(part 1 of 2)
# Autodesk Inventor assembly: Ensamblaje SCARA
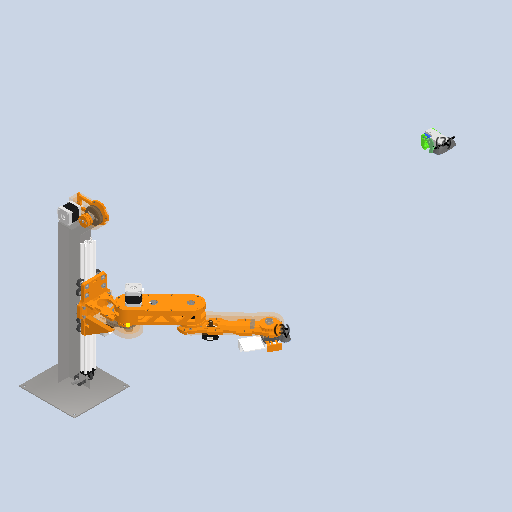
[picture p0: Inventor's stored thumbnail of the model, 512x512]
Saved by Autodesk Inventor 2026 (Build 300175050, 175E)
## iProperties
Created: 2025-07-17
Part Number: Ensamblaje SCARA
Document SubType Name: Assembly
Designer: bello
Mass: 5040.16 g
Surface Area: 9503.65 cm^2
Volume: 2049.58 cm^3
Density: 2.45911 g/cm^3
Author: bello
## Documents named in this file (71)
- A:\Federico Bellomi\UNLZ\5. Quinto Año\Proyecto Final\Ensamblaje\Ensamblaje SCARA.iam
- A:\Federico Bellomi\UNLZ\5. Quinto Año\Proyecto Final\Ensamblaje\Eje Z\Poste.ipt
- A:\Federico Bellomi\UNLZ\5. Quinto Año\Proyecto Final\Ensamblaje\Eje Z\Perfil 2040 200 mm v4.ipt
- A:\Federico Bellomi\UNLZ\5. Quinto Año\Proyecto Final\Ensamblaje\Eje Z\Tapa perfil de aluminio.ipt
- A:\Federico Bellomi\UNLZ\5. Quinto Año\Proyecto Final\Ensamblaje\download\Nema+17+Motor+Assembled\Nema+17+Motor+Assembled\Nema+17+Motor+Assembled.iam
- A:\Federico Bellomi\UNLZ\5. Quinto Año\Proyecto Final\Ensamblaje\Primer Segmento\Rueda v.ipt
- C:\Users\bello\OneDrive\Documentos\Inventor\Content Center Files\R2026\es-ES\DIN 625 SKF(1)\DIN 625 SKF - SKF 625-Z.ipt
- A:\Federico Bellomi\UNLZ\5. Quinto Año\Proyecto Final\Ensamblaje\download\Nema+17+Motor+Assembled\Engranaje para nema 17.ipt
- C:\Users\bello\OneDrive\Documentos\Inventor\Content Center Files\R2026\es-ES\DIN 625 SKF(1)\DIN 625 SKF - SKF 608-Z.ipt
- A:\Federico Bellomi\UNLZ\5. Quinto Año\Proyecto Final\Ensamblaje\Primer Segmento\Primer segmento - superior v1.2.ipt
- A:\Federico Bellomi\UNLZ\5. Quinto Año\Proyecto Final\Ensamblaje\Eje Z\Engranaje Insertado en pin.ipt
- C:\Users\bello\OneDrive\Documentos\Inventor\Content Center Files\R2026\es-ES\ISO 4014(2)\ISO 4014 - M5 x 35 - ISO.ipt
- C:\Users\bello\OneDrive\Documentos\Inventor\Content Center Files\R2026\es-ES\ISO 4014(2)\ISO 4014 - M8 x 50 - ISO.ipt
- C:\Users\bello\OneDrive\Documentos\Inventor\Content Center Files\R2026\es-ES\ISO 7089\ISO 7089 - 8 - 140 HV(1).ipt
- C:\Users\bello\OneDrive\Documentos\Inventor\Content Center Files\R2026\es-ES\ISO 7093 A\ISO 7093 A - ST 5 - 140 HV .ipt
- C:\Users\bello\OneDrive\Documentos\Inventor\Content Center Files\R2026\es-ES\ISO 4032(2)\ISO 4032 - M6 - ISO.ipt
- C:\Users\bello\OneDrive\Documentos\Inventor\Content Center Files\R2026\es-ES\ISO 4032(2)\ISO 4032 - M8 - ISO.ipt
- A:\Federico Bellomi\UNLZ\5. Quinto Año\Proyecto Final\Ensamblaje\Primer Segmento\Buje paraVslot.ipt
- C:\Users\bello\OneDrive\Documentos\Inventor\Content Center Files\R2026\es-ES\ISO 4032(2)\ISO 4032 - M5 - ISO.ipt
- A:\Federico Bellomi\UNLZ\5. Quinto Año\Proyecto Final\Ensamblaje\Eje Z\Buje para UPN.ipt
- C:\Users\bello\OneDrive\Documentos\Inventor\Content Center Files\R2026\es-ES\KS B 2023\KS B 2023 - 688 - 8 x 16 x 4 - 1.351.ipt
- A:\Federico Bellomi\UNLZ\5. Quinto Año\Proyecto Final\Ensamblaje\Primer Segmento\Soporte del primer segmento.ipt
- A:\Federico Bellomi\UNLZ\5. Quinto Año\Proyecto Final\Ensamblaje\Eje Z\Cono interno - Engranaje 1 eje Z.ipt
- A:\Federico Bellomi\UNLZ\5. Quinto Año\Proyecto Final\Ensamblaje\Eje Z\Engranaje 1 - Reductor Eje Z.ipt
- C:\Users\bello\OneDrive\Documentos\Inventor\Content Center Files\R2026\es-ES\BS 290 SKF(09)\BS 290 SKF - SKF 608-2Z.ipt
- C:\Users\bello\OneDrive\Documentos\Inventor\Content Center Files\R2026\es-ES\ISO 2338(2)\ISO 2338 - 8 h8 x 60.ipt
- C:\Users\bello\OneDrive\Documentos\Inventor\Content Center Files\R2026\es-ES\ISO 4032(2)\ISO 4032 - M3 - ISO.ipt
- A:\Federico Bellomi\UNLZ\5. Quinto Año\Proyecto Final\Ensamblaje\Eje Z\Caja reductora - eje z.ipt
- C:\Users\bello\OneDrive\Documentos\Inventor\Content Center Files\R2026\es-ES\ISO 4014(2)\ISO 4014 - M6 x 30 - ISO.ipt
- C:\Users\bello\OneDrive\Documentos\Inventor\Content Center Files\R2026\es-ES\ISO 7089\ISO 7089 - 6 - 140 HV(1).ipt
- A:\Federico Bellomi\UNLZ\5. Quinto Año\Proyecto Final\Ensamblaje\Eje Z\Tapa de caja reductora - eje z.ipt
- C:\Users\bello\OneDrive\Documentos\Inventor\Content Center Files\R2026\es-ES\ISO 4017(1)\ISO 4017 - M3 x 16 - ISO.ipt
- C:\Users\bello\OneDrive\Documentos\Inventor\Content Center Files\R2026\es-ES\ISO 7089\ISO 7089 - 3 - 140 HV(1).ipt
- A:\Federico Bellomi\UNLZ\5. Quinto Año\Proyecto Final\Ensamblaje\Eje Z\Engranaje 2 reductor Eje Z.ipt
- A:\Federico Bellomi\UNLZ\5. Quinto Año\Proyecto Final\Ensamblaje\Eje Z\Cono interno - Engranaje 2 eje Z.ipt
- A:\Federico Bellomi\UNLZ\5. Quinto Año\Proyecto Final\Ensamblaje\Primer Segmento\Engrajane doble - primer segmento.ipt
- A:\Federico Bellomi\UNLZ\5. Quinto Año\Proyecto Final\Ensamblaje\Primer Segmento\Engranaje simple - primer segmento.ipt
- A:\Federico Bellomi\UNLZ\5. Quinto Año\Proyecto Final\Ensamblaje\Primer Segmento\Segmento inferior.ipt
- C:\Users\bello\OneDrive\Documentos\Inventor\Content Center Files\R2026\es-ES\ISO 2338(2)\ISO 2338 - 8 h8 x 40.ipt
- A:\Federico Bellomi\UNLZ\5. Quinto Año\Proyecto Final\Ensamblaje\Primer Segmento\Polea Lisa - eje3mm.ipt
- C:\Users\bello\OneDrive\Documentos\Inventor\Content Center Files\R2026\es-ES\ISO 4014(2)\ISO 4014 - M3 x 20 - ISO.ipt
- C:\Users\bello\OneDrive\Documentos\Inventor\Content Center Files\R2026\es-ES\ISO 7045  H\ISO 7045 - M3 x 10_ - 4.8 - H - ISO.ipt
- C:\Users\bello\OneDrive\Documentos\Inventor\Content Center Files\R2026\es-ES\ISO 4017(1)\ISO 4017 - M5 x 25 - ISO.ipt
- C:\Users\bello\OneDrive\Documentos\Inventor\Content Center Files\R2026\es-ES\ISO 7089\ISO 7089 - 5 - 140 HV(1).ipt
- C:\Users\bello\OneDrive\Documentos\Inventor\Content Center Files\R2026\es-ES\JIS B 1521\JIS B 1521 - 6805 25x37x7x4.5.ipt
- C:\Users\bello\OneDrive\Documentos\Inventor\Content Center Files\R2026\es-ES\ISO 4017(1)\ISO 4017 - M4 x 40 - ISO.ipt
- C:\Users\bello\OneDrive\Documentos\Inventor\Content Center Files\R2026\es-ES\ISO 4032(2)\ISO 4032 - M4 - ISO.ipt
- C:\Users\bello\OneDrive\Documentos\Inventor\Content Center Files\R2026\es-ES\ISO 7045  H\ISO 7045 - M3 x 8_ - 4.8 - H - ISO.ipt
- A:\Federico Bellomi\UNLZ\5. Quinto Año\Proyecto Final\Ensamblaje\Segundo Segmento\Segundo segmento - superior.ipt
- A:\Federico Bellomi\UNLZ\5. Quinto Año\Proyecto Final\Ensamblaje\Segundo Segmento\Segundo segmento - inferior - Shape generator prueba 2 - 40%.ipt
- C:\Users\bello\OneDrive\Documentos\Inventor\Content Center Files\R2026\es-ES\ISO 7045  H\ISO 7045 - M4 x 16_ - 4.8 - H - ISO.ipt
- C:\Users\bello\OneDrive\Documentos\Inventor\Content Center Files\R2026\es-ES\ISO 7089\ISO 7089 - 4 - 140 HV(1).ipt
- A:\Federico Bellomi\UNLZ\5. Quinto Año\Proyecto Final\Ensamblaje\Segundo Segmento\Engranaje simple - segundo segmento.ipt
- A:\Federico Bellomi\UNLZ\5. Quinto Año\Proyecto Final\Ensamblaje\Segundo Segmento\Joint - Segundo segmento.ipt
- A:\Federico Bellomi\UNLZ\5. Quinto Año\Proyecto Final\Ensamblaje\Tercer Segmento\Tercer Segmento - inferior.ipt
- A:\Federico Bellomi\UNLZ\5. Quinto Año\Proyecto Final\Ensamblaje\Tercer Segmento\Tercer segmento - superior.ipt
- A:\Federico Bellomi\UNLZ\5. Quinto Año\Proyecto Final\Ensamblaje\Tercer Segmento\nema17_pancake\nema17_pancake\nema17_pancake.ipt
- A:\Federico Bellomi\UNLZ\5. Quinto Año\Proyecto Final\Ensamblaje\Primer Segmento\Joint - Primer segmento.ipt
- C:\Users\bello\OneDrive\Documentos\Inventor\Content Center Files\R2026\es-ES\ISO 2338(2)\ISO 2338 - 8 h8 x 50.ipt
- C:\Users\bello\OneDrive\Documentos\Inventor\Content Center Files\R2026\es-ES\ISO 2338(2)\ISO 2338 - 8 h8 x 30.ipt
- A:\Federico Bellomi\UNLZ\5. Quinto Año\Proyecto Final\Ensamblaje\Gripper\Base - Gripper.ipt
- A:\Federico Bellomi\UNLZ\5. Quinto Año\Proyecto Final\pince-robot-sg90-gripper-1.snapshot.26\Pince robot SG90\roue dentée 38A1\roue dentée 38A1\roue dentée 38A1.ipt
- A:\Federico Bellomi\UNLZ\5. Quinto Año\Proyecto Final\pince-robot-sg90-gripper-1.snapshot.26\Pince robot SG90\roue dentée 38B1\roue dentée 38B1\roue dentée 38B1.ipt
- A:\Federico Bellomi\UNLZ\5. Quinto Año\Proyecto Final\Ensamblaje\Gripper\Servo SG90\Servo SG90\Servo SG90.ipt
- A:\Federico Bellomi\UNLZ\5. Quinto Año\Proyecto Final\Ensamblaje\Gripper\logitech-c270-webcam-1.snapshot.1\Logitech c270\Logitech c270\Logitech c270.ipt
- A:\Federico Bellomi\UNLZ\5. Quinto Año\Proyecto Final\Ensamblaje\Gripper\Base - version 2.ipt
- A:\Federico Bellomi\UNLZ\5. Quinto Año\Proyecto Final\Ensamblaje\Gripper\logitech-c270-webcam-1.snapshot.1\Logitech c270\Round_gear.ipt
- A:\Federico Bellomi\UNLZ\5. Quinto Año\Proyecto Final\Ensamblaje\Gripper\Tapa - Gripper.ipt
- A:\Federico Bellomi\UNLZ\5. Quinto Año\Proyecto Final\Ensamblaje\Gripper\Pata Izquierda - versión 3.ipt
- A:\Federico Bellomi\UNLZ\5. Quinto Año\Proyecto Final\Ensamblaje\Gripper\Pata derecha - versión 3.ipt
- A:\Federico Bellomi\UNLZ\5. Quinto Año\Proyecto Final\Ensamblaje\Gripper\Base Marcador ECU + Gripper.ipt
## Components (260 placed, 70 different names)
1. Poste:1 — Coincidencia:1, Nivelación:1, Coincidencia:287, Coincidencia:288, Coincidencia:290, Coincidencia:484, Ángulo:3, Coincidencia:507, Ángulo:4, Coincidencia:508, Coincidencia:515, Ángulo:28, Ángulo:29
2. Perfil 2040 200 mm v4:2 — Insertar:1, Insertar:2, Coincidencia:424
3. Perfil 2040 200 mm v4:3 — Insertar:1, Coincidencia:1, Nivelación:1, Insertar:2, Coincidencia:1235, Nivelación:138
4. Rueda v:9
5. DIN 625 SKF- con escudo Z SKF 625-Z:18
6. DIN 625 SKF- con escudo Z SKF 625-Z:19
7. ISO 4014 M5 x 35:1 — Coincidencia:137, Coincidencia:138, Coincidencia:142, Coincidencia:143
8. ISO 7093 A ST 5 - 140 HV - A:1 — Coincidencia:138, Coincidencia:144
9. ISO 7093 A ST 5 - 140 HV - A:2 — Coincidencia:137, Coincidencia:142
10. ISO 4032 M6:1 — Coincidencia:143, Coincidencia:144
11. ISO 4014 M8 x 50:1 — Coincidencia:282, Coincidencia:283, Coincidencia:287, Coincidencia:289, Coincidencia:295, Coincidencia:297, Coincidencia:299
12. ISO 7089 8:1 — Coincidencia:282, Coincidencia:283, Coincidencia:288
13. ISO 7089 8:2 — Coincidencia:289, Coincidencia:290, Coincidencia:298
14. Buje para UPN:1 — Coincidencia:296, Coincidencia:297, Coincidencia:298
15. ISO 4032 M8:1 — Coincidencia:299, Coincidencia:300
16. KS B 2023 688 - 8 x 16 x 4:3 — Coincidencia:292, Coincidencia:293, Coincidencia:296
17. Engranaje Insertado en pin:1 — Coincidencia:291, Coincidencia:292, Coincidencia:293, Coincidencia:294, Coincidencia:295
18. KS B 2023 688 - 8 x 16 x 4:4 — Coincidencia:291, Coincidencia:294, Coincidencia:300
19. Tapa perfil de aluminio:1 — Coincidencia:424
20. ISO 2338 8 h8 x 60:1 — Coincidencia:469, Nivelación:62, Coincidencia:536, Coincidencia:551
21. BS 290 SKF- con dos escudos Z SKF 608-2Z:3 — Coincidencia:467, Coincidencia:469, Coincidencia:518, Nivelación:70
22. BS 290 SKF- con dos escudos Z SKF 608-2Z:4 — Coincidencia:467, Nivelación:62, Coincidencia:490, Nivelación:65, Coincidencia:537
23. Nema+17+Motor+Assembled:2 [sub-assembly] — Ángulo:3, Coincidencia:516, Coincidencia:517
24. ISO 4014 M6 x 30:1 — Nivelación:63, Coincidencia:509, Coincidencia:511, Coincidencia:514
25. ISO 4014 M6 x 30:2 — Nivelación:63, Coincidencia:481, Coincidencia:482, Coincidencia:510
26. ISO 4032 M6:2 — Coincidencia:481, Coincidencia:487
27. ISO 7089 6:2 — Coincidencia:482, Coincidencia:484, Coincidencia:487
28. Tapa de caja reductora - eje z:1 — Coincidencia:490, Nivelación:65, Coincidencia:519, Coincidencia:694, Coincidencia:695, Coincidencia:696, Coincidencia:697, Coincidencia:698, Coincidencia:699, Coincidencia:700, Coincidencia:701
29. ISO 4032 M6:3 — Coincidencia:512, Coincidencia:513
30. ISO 7089 6:3 — Coincidencia:512, Coincidencia:513, Coincidencia:514, Coincidencia:515
31. Caja reductora - eje z:1 — Coincidencia:507, Ángulo:4, Coincidencia:508, Coincidencia:509, Coincidencia:510, Coincidencia:511, Coincidencia:516, Coincidencia:517, Coincidencia:518, Nivelación:70, Coincidencia:519, Coincidencia:552
32. Engranaje 1 - Reductor Eje Z:2
33. Cono interno - Engranaje 1 eje Z:2 — Coincidencia:536, Coincidencia:537
34. ISO 4032 M3:3
35. ISO 4032 M3:4
36. ISO 4017 M3 x 16:3
37. ISO 4017 M3 x 16:4
38. ISO 7089 3:3
39. ISO 7089 3:4
40. Engranaje 2 reductor Eje Z:1 — Coincidencia:538, Coincidencia:539, Coincidencia:540, Coincidencia:541, Nivelación:78, Coincidencia:542, Nivelación:79, Ángulo:5, Ángulo:6
41. Cono interno - Engranaje 2 eje Z:1 — Coincidencia:538, Coincidencia:539, Coincidencia:540, Coincidencia:543, Coincidencia:545, Coincidencia:547, Coincidencia:549, Coincidencia:551, Coincidencia:552
42. ISO 4017 M3 x 16:5 — Coincidencia:543, Coincidencia:544, Coincidencia:550
43. ISO 7089 3:5 — Coincidencia:544, Coincidencia:549, Coincidencia:550
44. ISO 4032 M3:5 — Coincidencia:541, Nivelación:78, Ángulo:5
45. ISO 4032 M3:6 — Coincidencia:542, Nivelación:79, Ángulo:6
46. ISO 7089 3:6 — Coincidencia:546, Coincidencia:547, Coincidencia:548
47. ISO 4017 M3 x 16:6 — Coincidencia:545, Coincidencia:546, Coincidencia:548
48. ISO 7045 H M3 x 10 - 4.8 - H:1 — Coincidencia:697, Coincidencia:699
49. ISO 7045 H M3 x 10 - 4.8 - H:2 — Coincidencia:695, Coincidencia:700
50. ISO 7045 H M3 x 10 - 4.8 - H:3 — Coincidencia:696, Coincidencia:698
51. ISO 7045 H M3 x 10 - 4.8 - H:4 — Coincidencia:694, Coincidencia:701
52. ISO 2338 8 h8 x 40:3 — Coincidencia:901, Nivelación:110, Coincidencia:917
53. DIN 625 SKF- con escudo Z SKF 608-Z:5 — Coincidencia:895, Nivelación:107, Coincidencia:897
54. Engrajane doble - primer segmento:2 — Coincidencia:917, Nivelación:113, Nivelación:114
55. DIN 625 SKF- con escudo Z SKF 608-Z:6 — Coincidencia:899, Nivelación:108, Coincidencia:901, Nivelación:110
56. DIN 625 SKF- con escudo Z SKF 608-Z:9 — Coincidencia:900, Nivelación:109, Coincidencia:1197, Nivelación:133
57. Rueda v:28
58. DIN 625 SKF- con escudo Z SKF 625-Z:56
59. DIN 625 SKF- con escudo Z SKF 625-Z:57
60. ISO 4014 M5 x 35:21
61. Buje paraVslot:20
62. Rueda v:29
63. DIN 625 SKF- con escudo Z SKF 625-Z:58
64. DIN 625 SKF- con escudo Z SKF 625-Z:59
65. ISO 4014 M5 x 35:22
66. Buje paraVslot:21
67. ISO 4032 M5:22
68. ISO 7093 A ST 5 - 140 HV - A:28
69. ISO 4032 M5:23
70. ISO 7093 A ST 5 - 140 HV - A:29
71. Soporte del primer segmento:2 — Coincidencia:881, Coincidencia:882, Coincidencia:883, Coincidencia:884, Coincidencia:885, Coincidencia:886, Coincidencia:888, Ángulo:29, Coincidencia:1235, Nivelación:138
72. ISO 7093 A ST 5 - 140 HV - A:30
73. ISO 7093 A ST 5 - 140 HV - A:31
74. Rueda v:30
75. DIN 625 SKF- con escudo Z SKF 625-Z:60
76. DIN 625 SKF- con escudo Z SKF 625-Z:61
77. ISO 4014 M5 x 35:23
78. Buje paraVslot:22
79. ISO 4032 M5:24
80. ISO 7093 A ST 5 - 140 HV - A:32
81. ISO 7093 A ST 5 - 140 HV - A:33
82. Rueda v:31
83. DIN 625 SKF- con escudo Z SKF 625-Z:62
84. DIN 625 SKF- con escudo Z SKF 625-Z:63
85. ISO 4014 M5 x 35:24
86. Buje paraVslot:23
87. ISO 4032 M5:25
88. ISO 7093 A ST 5 - 140 HV - A:34
89. ISO 7093 A ST 5 - 140 HV - A:35
90. Engranaje para nema 17:4 — Coincidencia:903, Nivelación:114
91. Rueda v:32
92. DIN 625 SKF- con escudo Z SKF 625-Z:64
93. DIN 625 SKF- con escudo Z SKF 625-Z:65
94. ISO 4014 M5 x 35:25
95. Buje paraVslot:24
96. ISO 4032 M5:26
97. ISO 7093 A ST 5 - 140 HV - A:36
98. Rueda v:33
99. DIN 625 SKF- con escudo Z SKF 625-Z:66
100. DIN 625 SKF- con escudo Z SKF 625-Z:67
101. ISO 4014 M5 x 35:26
102. Buje paraVslot:25
103. ISO 4032 M5:27
104. ISO 7093 A ST 5 - 140 HV - A:37
105. Rueda v:34
106. DIN 625 SKF- con escudo Z SKF 625-Z:68
107. DIN 625 SKF- con escudo Z SKF 625-Z:69
108. ISO 4014 M5 x 35:27
109. Buje paraVslot:26
110. ISO 4032 M5:28
111. ISO 7093 A ST 5 - 140 HV - A:38
112. Rueda v:35
113. DIN 625 SKF- con escudo Z SKF 625-Z:70
114. DIN 625 SKF- con escudo Z SKF 625-Z:71
115. ISO 4014 M5 x 35:28
116. Buje paraVslot:27
117. ISO 4032 M5:29
118. ISO 7093 A ST 5 - 140 HV - A:39
119. ISO 4017 M5 x 25:5 — Coincidencia:884, Coincidencia:887, Ángulo:24
120. ISO 4017 M5 x 25:6 — Coincidencia:886, Ángulo:26, Coincidencia:890
121. ISO 4017 M5 x 25:7 — Coincidencia:885, Ángulo:27, Coincidencia:889
122. ISO 4017 M5 x 25:8 — Coincidencia:883, Ángulo:25, Coincidencia:891
123. ISO 4032 M5:30
124. ISO 4032 M5:31
125. ISO 4032 M5:32
126. ISO 4032 M5:33
127. ISO 7089 5:5
128. ISO 7089 5:6
129. ISO 7089 5:7
130. ISO 7089 5:8
131. Segmento inferior:1 — Coincidencia:881, Coincidencia:882, Coincidencia:887, Ángulo:24, Ángulo:25, Coincidencia:888, Ángulo:26, Ángulo:27, Coincidencia:889, Coincidencia:890, Coincidencia:891, Ángulo:28, Coincidencia:892, Coincidencia:893, Coincidencia:894, Coincidencia:895, Nivelación:107, Coincidencia:896, Coincidencia:898, Coincidencia:900, Nivelación:109
132. Nema+17+Motor+Assembled:5 [sub-assembly] — Coincidencia:892, Coincidencia:893, Coincidencia:894, Coincidencia:903
133. Primer segmento - superior v1.2:1 — Coincidencia:896, Coincidencia:897, Coincidencia:898, Coincidencia:899, Nivelación:108, Coincidencia:904, Coincidencia:905, Coincidencia:906, Coincidencia:907, Coincidencia:908, Coincidencia:909, Coincidencia:910, Coincidencia:911, Coincidencia:912, Coincidencia:913, Coincidencia:914, Coincidencia:915, Coincidencia:916, Nivelación:112, Coincidencia:1039, Coincidencia:1041
134. JIS B 1521 6805 25x37x7:3 — Coincidencia:916, Nivelación:112, Coincidencia:919
135. Engranaje simple - primer segmento:1 — Coincidencia:919, Nivelación:113, Coincidencia:929, Coincidencia:930, Coincidencia:931, Coincidencia:932, Coincidencia:1042, Coincidencia:1043, Coincidencia:1044, Coincidencia:1045
136. ISO 4017 M4 x 40:1 — Coincidencia:931, Coincidencia:935, Coincidencia:1043
137. ISO 4017 M4 x 40:2 — Coincidencia:930, Coincidencia:934, Coincidencia:1042
138. ISO 4017 M4 x 40:3 — Coincidencia:932, Coincidencia:936, Coincidencia:1045, Coincidencia:1184
139. ISO 4017 M4 x 40:4 — Coincidencia:929, Coincidencia:933, Coincidencia:1044
140. ISO 7045 H M3 x 8 - 4.8 - H:14 — Coincidencia:904, Coincidencia:910
141. ISO 7045 H M3 x 8 - 4.8 - H:15 — Coincidencia:909, Coincidencia:911
142. ISO 4032 M4:1 — Coincidencia:935, Coincidencia:1046
143. ISO 4032 M4:2 — Coincidencia:936, Coincidencia:1048
144. ISO 4032 M4:3 — Coincidencia:933, Coincidencia:1049
145. ISO 4032 M4:4 — Coincidencia:934, Coincidencia:1047
146. ISO 7045 H M3 x 8 - 4.8 - H:16 — Coincidencia:905, Coincidencia:912
147. ISO 7045 H M3 x 8 - 4.8 - H:17 — Coincidencia:908, Coincidencia:915
148. ISO 7045 H M3 x 8 - 4.8 - H:18 — Coincidencia:906, Coincidencia:913
149. ISO 7045 H M3 x 8 - 4.8 - H:19 — Coincidencia:907, Coincidencia:914
150. Segundo segmento - inferior - Shape generator prueba 2 - 40%:1 — Coincidencia:944, Coincidencia:945, Coincidencia:946, Coincidencia:947, Coincidencia:948, Coincidencia:949, Coincidencia:962, Coincidencia:963, Coincidencia:964, Coincidencia:965, Coincidencia:966, Coincidencia:967, Coincidencia:980, Coincidencia:981, Coincidencia:982, Nivelación:122, Coincidencia:1016, Coincidencia:1038, Coincidencia:1040, Coincidencia:1041, Coincidencia:1063, Coincidencia:1143, Coincidencia:1144, Coincidencia:1145, Coincidencia:1233, Coincidencia:1234
151. ISO 7045 H M4 x 16 - 4.8 - H:1 — Coincidencia:947, Coincidencia:958, Coincidencia:971, Coincidencia:1053, Coincidencia:1057
152. ISO 7045 H M4 x 16 - 4.8 - H:2 — Coincidencia:948, Coincidencia:961, Coincidencia:972, Coincidencia:1052, Coincidencia:1061
153. ISO 7045 H M4 x 16 - 4.8 - H:3 — Coincidencia:946, Coincidencia:957, Coincidencia:970, Coincidencia:1051, Coincidencia:1058
154. ISO 7045 H M4 x 16 - 4.8 - H:4 — Coincidencia:944, Coincidencia:955, Coincidencia:969, Coincidencia:1054, Coincidencia:1059
155. ISO 7045 H M4 x 16 - 4.8 - H:5 — Coincidencia:945, Coincidencia:956, Coincidencia:968, Coincidencia:1055, Coincidencia:1060
156. ISO 7045 H M4 x 16 - 4.8 - H:6 — Coincidencia:949, Coincidencia:959, Coincidencia:973, Coincidencia:1050, Coincidencia:1056
157. ISO 4032 M4:5 — Coincidencia:968, Coincidencia:977
158. ISO 4032 M4:6 — Coincidencia:969, Coincidencia:978
159. ISO 4032 M4:7 — Coincidencia:970, Coincidencia:975
160. ISO 4032 M4:8 — Coincidencia:971, Coincidencia:979
161. ISO 7089 4:1 — Coincidencia:957, Coincidencia:964
162. ISO 7089 4:2 — Coincidencia:955, Coincidencia:967, Coincidencia:978
163. ISO 7089 4:3 — Coincidencia:956, Coincidencia:966, Coincidencia:977
164. ISO 7089 4:4 — Coincidencia:958, Coincidencia:965, Coincidencia:975, Coincidencia:979
165. ISO 7089 4:5 — Coincidencia:959, Coincidencia:962
166. ISO 7089 4:6 — Coincidencia:961, Coincidencia:963, Coincidencia:974, Coincidencia:976
167. ISO 4032 M4:9 — Coincidencia:972, Coincidencia:976
168. ISO 4032 M4:10 — Coincidencia:973, Coincidencia:974
169. Segundo segmento - superior:1 — Coincidencia:980, Coincidencia:981, Coincidencia:982, Coincidencia:983, Coincidencia:984, Coincidencia:985, Coincidencia:987, Nivelación:115, Coincidencia:988, Nivelación:116, Coincidencia:1000, Coincidencia:1001, Coincidencia:1002, Coincidencia:1003, Coincidencia:1004, Coincidencia:1005, Coincidencia:1006, Coincidencia:1007, Coincidencia:1008, Coincidencia:1009, Coincidencia:1010, Coincidencia:1011, Coincidencia:1012, Coincidencia:1013, Coincidencia:1014, Coincidencia:1015, Coincidencia:1062
170. Engranaje para nema 17:5 — Coincidencia:986, Nivelación:119
171. DIN 625 SKF- con escudo Z SKF 608-Z:10 — Coincidencia:987, Nivelación:115, Coincidencia:989, Nivelación:117
172. DIN 625 SKF- con escudo Z SKF 608-Z:11 — Coincidencia:988, Nivelación:116, Coincidencia:1198, Nivelación:134
173. Engrajane doble - primer segmento:3 — Coincidencia:990, Nivelación:119, Nivelación:123
174. ISO 2338 8 h8 x 40:4 — Coincidencia:989, Nivelación:117, Coincidencia:990
175. Nema+17+Motor+Assembled:6 [sub-assembly] — Coincidencia:983, Coincidencia:984, Coincidencia:985, Coincidencia:986
176. ISO 4017 M4 x 40:5 — Coincidencia:1025, Coincidencia:1071, Coincidencia:1078
177. ISO 4017 M4 x 40:6 — Coincidencia:1027, Coincidencia:1073, Coincidencia:1076
178. ISO 4017 M4 x 40:7 — Coincidencia:1024, Coincidencia:1074, Coincidencia:1077
179. ISO 4017 M4 x 40:8 — Coincidencia:1026, Coincidencia:1072, Coincidencia:1075
180. Engranaje simple - segundo segmento:1 — Coincidencia:1024, Coincidencia:1025, Coincidencia:1026, Coincidencia:1027, Nivelación:123, Coincidencia:1064, Coincidencia:1066, Coincidencia:1067
181. ISO 7045 H M3 x 8 - 4.8 - H:20 — Coincidencia:1000, Coincidencia:1013
182. ISO 7045 H M3 x 8 - 4.8 - H:21 — Coincidencia:1001, Coincidencia:1014
183. ISO 7045 H M3 x 8 - 4.8 - H:22 — Coincidencia:1002, Coincidencia:1009
184. ISO 7045 H M3 x 8 - 4.8 - H:23 — Coincidencia:1003, Coincidencia:1012
185. ISO 7045 H M3 x 8 - 4.8 - H:24 — Coincidencia:1004, Coincidencia:1011
186. ISO 7045 H M3 x 8 - 4.8 - H:25 — Coincidencia:1007, Coincidencia:1015
187. ISO 7045 H M3 x 8 - 4.8 - H:26 — Coincidencia:1006, Coincidencia:1008
188. ISO 7045 H M3 x 8 - 4.8 - H:27 — Coincidencia:1005, Coincidencia:1010
189. DIN 625 SKF- con escudo Z SKF 608-Z:12 — Nivelación:122, Coincidencia:1016
190. Tercer Segmento - inferior:1 — Coincidencia:1031, Coincidencia:1032, Coincidencia:1033, Coincidencia:1035, Coincidencia:1036, Coincidencia:1037, Coincidencia:1127, Coincidencia:1160, Coincidencia:1161, Coincidencia:1162, Nivelación:127, Coincidencia:1165, Coincidencia:1166, Ángulo:30, Coincidencia:1167, Coincidencia:1168, Coincidencia:1169, Coincidencia:1170, Coincidencia:1171, Coincidencia:1172, Coincidencia:1173, Coincidencia:1174, Coincidencia:1175, Coincidencia:1176, Coincidencia:1177, Coincidencia:1178, Coincidencia:1179, Coincidencia:1180, Coincidencia:1181, Coincidencia:1182, Coincidencia:1183, Coincidencia:1237
191. Tercer segmento - superior:1 — Coincidencia:1031, Coincidencia:1032, Coincidencia:1033, Coincidencia:1068, Coincidencia:1069, Coincidencia:1070, Coincidencia:1111, Coincidencia:1113, Coincidencia:1114, Coincidencia:1115, Coincidencia:1116, Coincidencia:1117, Coincidencia:1127, Coincidencia:1191, Nivelación:131
192. nema17_pancake:1 — Coincidencia:1035, Coincidencia:1036, Coincidencia:1037, Coincidencia:1126
193. Joint - Primer segmento:1 — Coincidencia:1038, Coincidencia:1039, Coincidencia:1040, Coincidencia:1046, Coincidencia:1047, Coincidencia:1048, Coincidencia:1049, Coincidencia:1050, Coincidencia:1051, Coincidencia:1052, Coincidencia:1053, Coincidencia:1054, Coincidencia:1055, Coincidencia:1056, Coincidencia:1057, Coincidencia:1058, Coincidencia:1059, Coincidencia:1060, Coincidencia:1061, Coincidencia:1184
194. JIS B 1521 6805 25x37x7:5 — Coincidencia:1062, Coincidencia:1063, Coincidencia:1064, Coincidencia:1065
195. Joint - Segundo segmento:1 — Coincidencia:1065, Coincidencia:1066, Coincidencia:1067, Coincidencia:1068, Coincidencia:1069, Coincidencia:1070, Coincidencia:1075, Coincidencia:1076, Coincidencia:1077, Coincidencia:1078, Coincidencia:1079, Coincidencia:1080, Coincidencia:1081, Coincidencia:1082, Coincidencia:1095, Coincidencia:1096, Coincidencia:1097, Coincidencia:1098, Coincidencia:1103, Coincidencia:1104, Coincidencia:1105, Coincidencia:1106, Coincidencia:1107, Coincidencia:1108, Coincidencia:1109, Coincidencia:1110
196. ISO 4032 M4:11 — Coincidencia:1073, Coincidencia:1081
197. ISO 4032 M4:12 — Coincidencia:1074, Coincidencia:1082
198. ISO 4032 M4:13 — Coincidencia:1072, Coincidencia:1079
199. ISO 4032 M4:14 — Coincidencia:1071, Coincidencia:1080
200. ISO 7045 H M4 x 16 - 4.8 - H:7 — Coincidencia:1098, Coincidencia:1105
201. ISO 7089 4:7 — Coincidencia:1114, Coincidencia:1120
202. ISO 4032 M4:15 — Coincidencia:1120
203. ISO 7045 H M4 x 16 - 4.8 - H:8 — Coincidencia:1097, Coincidencia:1106
204. ISO 7089 4:8 — Coincidencia:1115, Coincidencia:1119
205. ISO 4032 M4:16 — Coincidencia:1119
206. ISO 7045 H M4 x 16 - 4.8 - H:10 — Coincidencia:1104, Coincidencia:1110
207. ISO 7089 4:10 — Coincidencia:1111, Coincidencia:1112
208. ISO 4032 M4:18 — Coincidencia:1112
209. ISO 7045 H M4 x 16 - 4.8 - H:11 — Coincidencia:1096, Coincidencia:1108
210. ISO 7089 4:11 — Coincidencia:1116, Coincidencia:1118, Coincidencia:1122
211. ISO 4032 M4:19 — Coincidencia:1122
212. ISO 7045 H M4 x 16 - 4.8 - H:12 — Coincidencia:1095, Coincidencia:1107
213. ISO 7089 4:12 — Coincidencia:1117
214. ISO 4032 M4:20 — Coincidencia:1118
215. ISO 7045 H M4 x 16 - 4.8 - H:14 — Coincidencia:1103, Coincidencia:1109
216. ISO 7089 4:14 — Coincidencia:1113, Coincidencia:1121
217. ISO 4032 M4:22 — Coincidencia:1121
218. Engranaje para nema 17:6 — Coincidencia:1126, Nivelación:128
219. ISO 4014 M3 x 20:3 — Coincidencia:1233
220. Polea Lisa - eje3mm:3
221. ISO 4032 M3:11
222. ISO 4032 M3:12 — Coincidencia:1144
223. ISO 7089 3:9 — Coincidencia:1143, Coincidencia:1145, Coincidencia:1234
224. ISO 4014 M3 x 20:4 — Coincidencia:1160
225. Polea Lisa - eje3mm:4 — Nivelación:126
226. ISO 4032 M3:13
227. ISO 4032 M3:14 — Coincidencia:1167
228. ISO 7089 3:10 — Coincidencia:1165, Coincidencia:1237
229. ISO 4014 M3 x 20:5 — Coincidencia:1161
230. Polea Lisa - eje3mm:5 — Nivelación:126
231. ISO 4032 M3:15
232. ISO 4032 M3:16 — Coincidencia:1166, Ángulo:30
233. ISO 7089 3:11
234. Engranaje simple - segundo segmento:2 — Coincidencia:1163, Coincidencia:1164, Nivelación:128, Coincidencia:1222, Coincidencia:1223, Coincidencia:1236
235. JIS B 1521 6805 25x37x7:6 — Coincidencia:1162, Nivelación:127, Coincidencia:1163, Coincidencia:1164
236. ISO 7045 H M3 x 8 - 4.8 - H:28 — Coincidencia:1168, Coincidencia:1182
237. ISO 7045 H M3 x 8 - 4.8 - H:29 — Coincidencia:1169, Coincidencia:1180
238. ISO 7045 H M3 x 8 - 4.8 - H:30 — Coincidencia:1170, Coincidencia:1178
239. ISO 7045 H M3 x 8 - 4.8 - H:31 — Coincidencia:1171, Coincidencia:1176
240. ISO 7045 H M3 x 8 - 4.8 - H:32 — Coincidencia:1174, Coincidencia:1181
241. ISO 7045 H M3 x 8 - 4.8 - H:33 — Coincidencia:1175, Coincidencia:1183
242. ISO 7045 H M3 x 8 - 4.8 - H:34 — Coincidencia:1173, Coincidencia:1179
243. ISO 7045 H M3 x 8 - 4.8 - H:35 — Coincidencia:1172, Coincidencia:1177
244. DIN 625 SKF- con escudo Z SKF 608-Z:13 — Coincidencia:1191, Nivelación:131, Coincidencia:1199, Nivelación:135
245. ISO 2338 8 h8 x 50:1 — Coincidencia:1197, Nivelación:133
246. ISO 2338 8 h8 x 50:2 — Coincidencia:1198, Nivelación:134
247. ISO 2338 8 h8 x 30:1 — Coincidencia:1199, Nivelación:135
248. roue dentée 38A1:1 — Coincidencia:1213, Nivelación:136
249. roue dentée 38B1:1 — Coincidencia:1210
250. Base - Gripper:1 — Coincidencia:1207, Coincidencia:1208, Coincidencia:1209, Coincidencia:1210, Coincidencia:1211, Coincidencia:1212
251. Servo SG90:1 — Coincidencia:1207, Coincidencia:1208, Coincidencia:1209, Coincidencia:1213, Nivelación:136
252. Logitech c270:1 — Coincidencia:1211, Coincidencia:1212
253. Base - version 2:1 — Coincidencia:1214, Ángulo:31, Coincidencia:1215, Coincidencia:1217, Ángulo:32, Coincidencia:1218, Coincidencia:1219, Coincidencia:1220, Coincidencia:1221, Coincidencia:1228, Coincidencia:1229, Coincidencia:1230, Coincidencia:1231
254. Round_gear:1 — Coincidencia:1216, Nivelación:137
255. Servo SG90:2 — Coincidencia:1214, Ángulo:31, Coincidencia:1215, Coincidencia:1216, Nivelación:137
256. Logitech c270:2 — Coincidencia:1217, Ángulo:32, Coincidencia:1218
257. Tapa - Gripper:1 — Coincidencia:1219, Coincidencia:1220, Coincidencia:1221, Coincidencia:1222, Coincidencia:1223, Coincidencia:1236
258. Pata derecha - versión 3:1 — Coincidencia:1228, Coincidencia:1229
259. Pata Izquierda - versión 3:1 — Coincidencia:1230, Coincidencia:1231, Coincidencia:1232, Ángulo:33
260. Base Marcador ECU + Gripper:1 — Coincidencia:1232, Ángulo:33
## Relationships (552: Mate 480, Flush 52, Angle 18, Insert 2)
- Insertar:1: Perfil 2040 200 mm v4:2 ↔ Perfil 2040 200 mm v4:3
- Coincidencia:1 [Mate]: Poste:1 ↔ Perfil 2040 200 mm v4:3
- Nivelación:1 [Flush]: Poste:1 ↔ Perfil 2040 200 mm v4:3
- Insertar:2: Perfil 2040 200 mm v4:2 ↔ Perfil 2040 200 mm v4:3
- [Mate]: Rueda v:9 ↔ DIN 625 SKF- con escudo Z SKF 625-Z:18
- [Mate]: Rueda v:9 ↔ DIN 625 SKF- con escudo Z SKF 625-Z:19
- [Flush]: Rueda v:9 ↔ DIN 625 SKF- con escudo Z SKF 625-Z:18
- [Flush]: Rueda v:9 ↔ DIN 625 SKF- con escudo Z SKF 625-Z:19
- Coincidencia:137 [Mate]: ISO 4014 M5 x 35:1 ↔ ISO 7093 A ST 5 - 140 HV - A:2
- Coincidencia:138 [Mate]: ISO 4014 M5 x 35:1 ↔ ISO 7093 A ST 5 - 140 HV - A:1
- Coincidencia:142 [Mate]: ISO 4014 M5 x 35:1 ↔ ISO 7093 A ST 5 - 140 HV - A:2
- Coincidencia:143 [Mate]: ISO 4014 M5 x 35:1 ↔ ISO 4032 M6:1
- Coincidencia:144 [Mate]: ISO 7093 A ST 5 - 140 HV - A:1 ↔ ISO 4032 M6:1
- Coincidencia:282 [Mate]: ISO 4014 M8 x 50:1 ↔ ISO 7089 8:1
- Coincidencia:283 [Mate]: ISO 4014 M8 x 50:1 ↔ ISO 7089 8:1
- Coincidencia:287 [Mate]: Poste:1 ↔ ISO 4014 M8 x 50:1
- Coincidencia:288 [Mate]: Poste:1 ↔ ISO 7089 8:1
- Coincidencia:289 [Mate]: ISO 4014 M8 x 50:1 ↔ ISO 7089 8:2
- Coincidencia:290 [Mate]: Poste:1 ↔ ISO 7089 8:2
- Coincidencia:291 [Mate]: Engranaje Insertado en pin:1 ↔ KS B 2023 688 - 8 x 16 x 4:4
- Coincidencia:292 [Mate]: KS B 2023 688 - 8 x 16 x 4:3 ↔ Engranaje Insertado en pin:1
- Coincidencia:293 [Mate]: KS B 2023 688 - 8 x 16 x 4:3 ↔ Engranaje Insertado en pin:1
- Coincidencia:294 [Mate]: Engranaje Insertado en pin:1 ↔ KS B 2023 688 - 8 x 16 x 4:4
- Coincidencia:295 [Mate]: ISO 4014 M8 x 50:1 ↔ Engranaje Insertado en pin:1
- Coincidencia:296 [Mate]: Buje para UPN:1 ↔ KS B 2023 688 - 8 x 16 x 4:3
- Coincidencia:297 [Mate]: ISO 4014 M8 x 50:1 ↔ Buje para UPN:1
- Coincidencia:298 [Mate]: ISO 7089 8:2 ↔ Buje para UPN:1
- Coincidencia:299 [Mate]: ISO 4014 M8 x 50:1 ↔ ISO 4032 M8:1
- Coincidencia:300 [Mate]: ISO 4032 M8:1 ↔ KS B 2023 688 - 8 x 16 x 4:4
- Coincidencia:424 [Mate]: Perfil 2040 200 mm v4:2 ↔ Tapa perfil de aluminio:1
- Coincidencia:467 [Mate]: BS 290 SKF- con dos escudos Z SKF 608-2Z:3 ↔ BS 290 SKF- con dos escudos Z SKF 608-2Z:4
- Coincidencia:469 [Mate]: ISO 2338 8 h8 x 60:1 ↔ BS 290 SKF- con dos escudos Z SKF 608-2Z:3
- Nivelación:62 [Flush]: ISO 2338 8 h8 x 60:1 ↔ BS 290 SKF- con dos escudos Z SKF 608-2Z:4
- Nivelación:63 [Flush]: ISO 4014 M6 x 30:1 ↔ ISO 4014 M6 x 30:2
- Coincidencia:481 [Mate]: ISO 4014 M6 x 30:2 ↔ ISO 4032 M6:2
- Coincidencia:482 [Mate]: ISO 4014 M6 x 30:2 ↔ ISO 7089 6:2
- Coincidencia:484 [Mate]: Poste:1 ↔ ISO 7089 6:2
- Coincidencia:487 [Mate]: ISO 4032 M6:2 ↔ ISO 7089 6:2
- Coincidencia:490 [Mate]: BS 290 SKF- con dos escudos Z SKF 608-2Z:4 ↔ Tapa de caja reductora - eje z:1
- Ángulo:3 [Angle] (0 deg): Poste:1 ↔ Nema+17+Motor+Assembled:2
- Nivelación:65 [Flush]: BS 290 SKF- con dos escudos Z SKF 608-2Z:4 ↔ Tapa de caja reductora - eje z:1
- Coincidencia:507 [Mate]: Poste:1 ↔ Caja reductora - eje z:1
- Ángulo:4 [Angle] (0 deg): Poste:1 ↔ Caja reductora - eje z:1
- Coincidencia:508 [Mate]: Poste:1 ↔ Caja reductora - eje z:1
- Coincidencia:509 [Mate]: ISO 4014 M6 x 30:1 ↔ Caja reductora - eje z:1
- Coincidencia:510 [Mate]: ISO 4014 M6 x 30:2 ↔ Caja reductora - eje z:1
- Coincidencia:511 [Mate]: ISO 4014 M6 x 30:1 ↔ Caja reductora - eje z:1
- Coincidencia:512 [Mate]: ISO 4032 M6:3 ↔ ISO 7089 6:3
- Coincidencia:513 [Mate]: ISO 4032 M6:3 ↔ ISO 7089 6:3
- Coincidencia:514 [Mate]: ISO 4014 M6 x 30:1 ↔ ISO 7089 6:3
- Coincidencia:515 [Mate]: Poste:1 ↔ ISO 7089 6:3
- Coincidencia:516 [Mate]: Nema+17+Motor+Assembled:2 ↔ Caja reductora - eje z:1
- Coincidencia:517 [Mate]: Nema+17+Motor+Assembled:2 ↔ Caja reductora - eje z:1
- Coincidencia:518 [Mate]: BS 290 SKF- con dos escudos Z SKF 608-2Z:3 ↔ Caja reductora - eje z:1
- Nivelación:70 [Flush]: BS 290 SKF- con dos escudos Z SKF 608-2Z:3 ↔ Caja reductora - eje z:1
- Coincidencia:519 [Mate]: Tapa de caja reductora - eje z:1 ↔ Caja reductora - eje z:1
- [Mate]: Engranaje 1 - Reductor Eje Z:2 ↔ Cono interno - Engranaje 1 eje Z:2
- [Mate]: Engranaje 1 - Reductor Eje Z:2 ↔ Cono interno - Engranaje 1 eje Z:2
- [Mate]: Engranaje 1 - Reductor Eje Z:2 ↔ Cono interno - Engranaje 1 eje Z:2
- [Flush]: Engranaje 1 - Reductor Eje Z:2 ↔ ISO 4032 M3:4
- [Flush]: Engranaje 1 - Reductor Eje Z:2 ↔ ISO 4032 M3:3
- [Mate]: Cono interno - Engranaje 1 eje Z:2 ↔ ISO 4017 M3 x 16:3
- [Mate]: Cono interno - Engranaje 1 eje Z:2 ↔ ISO 4017 M3 x 16:4
- [Mate]: ISO 4017 M3 x 16:3 ↔ ISO 7089 3:3
- [Mate]: ISO 4017 M3 x 16:4 ↔ ISO 7089 3:4
- [Mate]: Cono interno - Engranaje 1 eje Z:2 ↔ ISO 7089 3:3
- [Mate]: Cono interno - Engranaje 1 eje Z:2 ↔ ISO 7089 3:4
- [Mate]: ISO 4017 M3 x 16:4 ↔ ISO 7089 3:4
- [Mate]: ISO 4017 M3 x 16:3 ↔ ISO 7089 3:3
- [Mate]: ISO 4032 M3:4 ↔ ISO 4017 M3 x 16:3
- [Mate]: ISO 4032 M3:3 ↔ ISO 4017 M3 x 16:4
- [Flush]: Engranaje 1 - Reductor Eje Z:2 ↔ ISO 4032 M3:3
- [Flush]: Engranaje 1 - Reductor Eje Z:2 ↔ ISO 4032 M3:4
- Coincidencia:536 [Mate]: ISO 2338 8 h8 x 60:1 ↔ Cono interno - Engranaje 1 eje Z:2
- Coincidencia:537 [Mate] (4 mm): BS 290 SKF- con dos escudos Z SKF 608-2Z:4 ↔ Cono interno - Engranaje 1 eje Z:2
- Coincidencia:538 [Mate]: Engranaje 2 reductor Eje Z:1 ↔ Cono interno - Engranaje 2 eje Z:1
- Coincidencia:539 [Mate]: Engranaje 2 reductor Eje Z:1 ↔ Cono interno - Engranaje 2 eje Z:1
- Coincidencia:540 [Mate]: Engranaje 2 reductor Eje Z:1 ↔ Cono interno - Engranaje 2 eje Z:1
- Coincidencia:541 [Mate]: Engranaje 2 reductor Eje Z:1 ↔ ISO 4032 M3:5
- Nivelación:78 [Flush]: Engranaje 2 reductor Eje Z:1 ↔ ISO 4032 M3:5
- Coincidencia:542 [Mate]: Engranaje 2 reductor Eje Z:1 ↔ ISO 4032 M3:6
- Nivelación:79 [Flush]: Engranaje 2 reductor Eje Z:1 ↔ ISO 4032 M3:6
- Ángulo:5 [Angle] (0 deg): Engranaje 2 reductor Eje Z:1 ↔ ISO 4032 M3:5
- Ángulo:6 [Angle] (0 deg): Engranaje 2 reductor Eje Z:1 ↔ ISO 4032 M3:6
- Coincidencia:543 [Mate]: Cono interno - Engranaje 2 eje Z:1 ↔ ISO 4017 M3 x 16:5
- Coincidencia:544 [Mate]: ISO 4017 M3 x 16:5 ↔ ISO 7089 3:5
- Coincidencia:545 [Mate]: Cono interno - Engranaje 2 eje Z:1 ↔ ISO 4017 M3 x 16:6
- Coincidencia:546 [Mate]: ISO 7089 3:6 ↔ ISO 4017 M3 x 16:6
- Coincidencia:547 [Mate]: Cono interno - Engranaje 2 eje Z:1 ↔ ISO 7089 3:6
- Coincidencia:548 [Mate]: ISO 7089 3:6 ↔ ISO 4017 M3 x 16:6
- Coincidencia:549 [Mate]: Cono interno - Engranaje 2 eje Z:1 ↔ ISO 7089 3:5
- Coincidencia:550 [Mate]: ISO 4017 M3 x 16:5 ↔ ISO 7089 3:5
- Coincidencia:551 [Mate]: ISO 2338 8 h8 x 60:1 ↔ Cono interno - Engranaje 2 eje Z:1
- Coincidencia:552 [Mate] (7 mm): Caja reductora - eje z:1 ↔ Cono interno - Engranaje 2 eje Z:1
- Coincidencia:694 [Mate]: Tapa de caja reductora - eje z:1 ↔ ISO 7045 H M3 x 10 - 4.8 - H:4
- Coincidencia:695 [Mate]: Tapa de caja reductora - eje z:1 ↔ ISO 7045 H M3 x 10 - 4.8 - H:2
- Coincidencia:696 [Mate]: Tapa de caja reductora - eje z:1 ↔ ISO 7045 H M3 x 10 - 4.8 - H:3
- Coincidencia:697 [Mate]: Tapa de caja reductora - eje z:1 ↔ ISO 7045 H M3 x 10 - 4.8 - H:1
- Coincidencia:698 [Mate]: Tapa de caja reductora - eje z:1 ↔ ISO 7045 H M3 x 10 - 4.8 - H:3
- Coincidencia:699 [Mate]: Tapa de caja reductora - eje z:1 ↔ ISO 7045 H M3 x 10 - 4.8 - H:1
- Coincidencia:700 [Mate]: Tapa de caja reductora - eje z:1 ↔ ISO 7045 H M3 x 10 - 4.8 - H:2
- Coincidencia:701 [Mate]: Tapa de caja reductora - eje z:1 ↔ ISO 7045 H M3 x 10 - 4.8 - H:4
- [Mate]: Rueda v:28 ↔ DIN 625 SKF- con escudo Z SKF 625-Z:56
- [Mate]: Rueda v:28 ↔ DIN 625 SKF- con escudo Z SKF 625-Z:57
- [Flush]: Rueda v:28 ↔ DIN 625 SKF- con escudo Z SKF 625-Z:56
- [Flush]: Rueda v:28 ↔ DIN 625 SKF- con escudo Z SKF 625-Z:57
- [Mate]: DIN 625 SKF- con escudo Z SKF 625-Z:56 ↔ ISO 4014 M5 x 35:21
- [Mate]: DIN 625 SKF- con escudo Z SKF 625-Z:56 ↔ ISO 4014 M5 x 35:21
- [Mate]: ISO 4014 M5 x 35:21 ↔ Buje paraVslot:20
- [Mate]: DIN 625 SKF- con escudo Z SKF 625-Z:57 ↔ Buje paraVslot:20
- [Mate]: Rueda v:29 ↔ DIN 625 SKF- con escudo Z SKF 625-Z:58
- [Mate]: Rueda v:29 ↔ DIN 625 SKF- con escudo Z SKF 625-Z:59
- [Flush]: Rueda v:29 ↔ DIN 625 SKF- con escudo Z SKF 625-Z:58
- [Flush]: Rueda v:29 ↔ DIN 625 SKF- con escudo Z SKF 625-Z:59
- [Mate]: DIN 625 SKF- con escudo Z SKF 625-Z:58 ↔ ISO 4014 M5 x 35:22
- [Mate]: DIN 625 SKF- con escudo Z SKF 625-Z:58 ↔ ISO 4014 M5 x 35:22
- [Mate]: ISO 4014 M5 x 35:22 ↔ Buje paraVslot:21
- [Mate]: DIN 625 SKF- con escudo Z SKF 625-Z:59 ↔ Buje paraVslot:21
- [Mate]: ISO 4014 M5 x 35:22 ↔ ISO 7093 A ST 5 - 140 HV - A:28
- [Mate]: ISO 4014 M5 x 35:22 ↔ ISO 4032 M5:22
- [Mate]: ISO 4014 M5 x 35:21 ↔ ISO 7093 A ST 5 - 140 HV - A:29
- [Mate]: ISO 4014 M5 x 35:21 ↔ ISO 4032 M5:23
- [Mate]: ISO 4032 M5:23 ↔ ISO 7093 A ST 5 - 140 HV - A:29
- [Mate]: ISO 4032 M5:22 ↔ ISO 7093 A ST 5 - 140 HV - A:28
- [Mate]: ISO 4014 M5 x 35:22 ↔ Soporte del primer segmento:2
- [Mate]: ISO 7093 A ST 5 - 140 HV - A:28 ↔ Soporte del primer segmento:2
- [Mate]: ISO 4014 M5 x 35:22 ↔ ISO 7093 A ST 5 - 140 HV - A:30
- [Mate]: Soporte del primer segmento:2 ↔ ISO 7093 A ST 5 - 140 HV - A:30
- [Mate]: Buje paraVslot:21 ↔ ISO 7093 A ST 5 - 140 HV - A:30
- [Mate]: ISO 4014 M5 x 35:21 ↔ Soporte del primer segmento:2
- [Mate]: ISO 4014 M5 x 35:21 ↔ ISO 7093 A ST 5 - 140 HV - A:31
- [Mate]: Soporte del primer segmento:2 ↔ ISO 7093 A ST 5 - 140 HV - A:31
- [Mate]: Buje paraVslot:20 ↔ ISO 7093 A ST 5 - 140 HV - A:31
- [Mate]: ISO 7093 A ST 5 - 140 HV - A:29 ↔ Soporte del primer segmento:2
- [Mate]: Rueda v:30 ↔ DIN 625 SKF- con escudo Z SKF 625-Z:60
- [Mate]: Rueda v:30 ↔ DIN 625 SKF- con escudo Z SKF 625-Z:61
- [Flush]: Rueda v:30 ↔ DIN 625 SKF- con escudo Z SKF 625-Z:60
- [Flush]: Rueda v:30 ↔ DIN 625 SKF- con escudo Z SKF 625-Z:61
- [Mate]: DIN 625 SKF- con escudo Z SKF 625-Z:60 ↔ ISO 4014 M5 x 35:23
- [Mate]: DIN 625 SKF- con escudo Z SKF 625-Z:60 ↔ ISO 4014 M5 x 35:23
- [Mate]: ISO 4014 M5 x 35:23 ↔ Buje paraVslot:22
- [Mate]: DIN 625 SKF- con escudo Z SKF 625-Z:61 ↔ Buje paraVslot:22
- [Mate]: ISO 4014 M5 x 35:23 ↔ ISO 7093 A ST 5 - 140 HV - A:32
- [Mate]: ISO 4014 M5 x 35:23 ↔ ISO 4032 M5:24
- [Mate]: ISO 4032 M5:24 ↔ ISO 7093 A ST 5 - 140 HV - A:32
- [Mate]: ISO 4014 M5 x 35:23 ↔ ISO 7093 A ST 5 - 140 HV - A:33
- [Mate]: Buje paraVslot:22 ↔ ISO 7093 A ST 5 - 140 HV - A:33
- [Mate]: Rueda v:31 ↔ DIN 625 SKF- con escudo Z SKF 625-Z:62
- [Mate]: Rueda v:31 ↔ DIN 625 SKF- con escudo Z SKF 625-Z:63
- [Flush]: Rueda v:31 ↔ DIN 625 SKF- con escudo Z SKF 625-Z:62
- [Flush]: Rueda v:31 ↔ DIN 625 SKF- con escudo Z SKF 625-Z:63
- [Mate]: DIN 625 SKF- con escudo Z SKF 625-Z:62 ↔ ISO 4014 M5 x 35:24
- [Mate]: DIN 625 SKF- con escudo Z SKF 625-Z:62 ↔ ISO 4014 M5 x 35:24
- [Mate]: ISO 4014 M5 x 35:24 ↔ Buje paraVslot:23
- [Mate]: DIN 625 SKF- con escudo Z SKF 625-Z:63 ↔ Buje paraVslot:23
- [Mate]: ISO 4014 M5 x 35:24 ↔ ISO 7093 A ST 5 - 140 HV - A:34
- [Mate]: ISO 4014 M5 x 35:24 ↔ ISO 4032 M5:25
- [Mate]: ISO 4032 M5:25 ↔ ISO 7093 A ST 5 - 140 HV - A:34
- [Mate]: ISO 4014 M5 x 35:24 ↔ ISO 7093 A ST 5 - 140 HV - A:35
- [Mate]: Buje paraVslot:23 ↔ ISO 7093 A ST 5 - 140 HV - A:35
- [Mate]: Soporte del primer segmento:2 ↔ ISO 4014 M5 x 35:24
- [Mate]: Soporte del primer segmento:2 ↔ ISO 7093 A ST 5 - 140 HV - A:34
- [Mate]: Soporte del primer segmento:2 ↔ ISO 7093 A ST 5 - 140 HV - A:35
- [Mate]: Soporte del primer segmento:2 ↔ ISO 4014 M5 x 35:23
- [Mate]: Soporte del primer segmento:2 ↔ ISO 7093 A ST 5 - 140 HV - A:32
- [Mate]: Soporte del primer segmento:2 ↔ ISO 7093 A ST 5 - 140 HV - A:33
- [Mate]: Rueda v:32 ↔ DIN 625 SKF- con escudo Z SKF 625-Z:64
- [Mate]: Rueda v:32 ↔ DIN 625 SKF- con escudo Z SKF 625-Z:65
- [Flush]: Rueda v:32 ↔ DIN 625 SKF- con escudo Z SKF 625-Z:64
- [Flush]: Rueda v:32 ↔ DIN 625 SKF- con escudo Z SKF 625-Z:65
- [Mate]: DIN 625 SKF- con escudo Z SKF 625-Z:64 ↔ ISO 4014 M5 x 35:25
- [Mate]: DIN 625 SKF- con escudo Z SKF 625-Z:64 ↔ ISO 4014 M5 x 35:25
- [Mate]: ISO 4014 M5 x 35:25 ↔ Buje paraVslot:24
- [Mate]: DIN 625 SKF- con escudo Z SKF 625-Z:65 ↔ Buje paraVslot:24
- [Mate]: ISO 4014 M5 x 35:25 ↔ ISO 4032 M5:26
- [Mate]: ISO 4014 M5 x 35:25 ↔ ISO 7093 A ST 5 - 140 HV - A:36
- [Mate]: Buje paraVslot:24 ↔ ISO 7093 A ST 5 - 140 HV - A:36
- [Mate]: Rueda v:33 ↔ DIN 625 SKF- con escudo Z SKF 625-Z:66
- [Mate]: Rueda v:33 ↔ DIN 625 SKF- con escudo Z SKF 625-Z:67
- [Flush]: Rueda v:33 ↔ DIN 625 SKF- con escudo Z SKF 625-Z:66
- [Flush]: Rueda v:33 ↔ DIN 625 SKF- con escudo Z SKF 625-Z:67
- [Mate]: DIN 625 SKF- con escudo Z SKF 625-Z:66 ↔ ISO 4014 M5 x 35:26
- [Mate]: DIN 625 SKF- con escudo Z SKF 625-Z:66 ↔ ISO 4014 M5 x 35:26
- [Mate]: ISO 4014 M5 x 35:26 ↔ Buje paraVslot:25
- [Mate]: DIN 625 SKF- con escudo Z SKF 625-Z:67 ↔ Buje paraVslot:25
- [Mate]: ISO 4014 M5 x 35:26 ↔ ISO 4032 M5:27
- [Mate]: ISO 4014 M5 x 35:26 ↔ ISO 7093 A ST 5 - 140 HV - A:37
- [Mate]: Buje paraVslot:25 ↔ ISO 7093 A ST 5 - 140 HV - A:37
- [Mate]: Rueda v:34 ↔ DIN 625 SKF- con escudo Z SKF 625-Z:68
- [Mate]: Rueda v:34 ↔ DIN 625 SKF- con escudo Z SKF 625-Z:69
- [Flush]: Rueda v:34 ↔ DIN 625 SKF- con escudo Z SKF 625-Z:68
- [Flush]: Rueda v:34 ↔ DIN 625 SKF- con escudo Z SKF 625-Z:69
- [Mate]: DIN 625 SKF- con escudo Z SKF 625-Z:68 ↔ ISO 4014 M5 x 35:27
- [Mate]: DIN 625 SKF- con escudo Z SKF 625-Z:68 ↔ ISO 4014 M5 x 35:27
- [Mate]: ISO 4014 M5 x 35:27 ↔ Buje paraVslot:26
- [Mate]: DIN 625 SKF- con escudo Z SKF 625-Z:69 ↔ Buje paraVslot:26
- [Mate]: ISO 4014 M5 x 35:27 ↔ ISO 4032 M5:28
- [Mate]: ISO 4014 M5 x 35:27 ↔ ISO 7093 A ST 5 - 140 HV - A:38
- [Mate]: Buje paraVslot:26 ↔ ISO 7093 A ST 5 - 140 HV - A:38
- [Mate]: Rueda v:35 ↔ DIN 625 SKF- con escudo Z SKF 625-Z:70
- [Mate]: Rueda v:35 ↔ DIN 625 SKF- con escudo Z SKF 625-Z:71
- [Flush]: Rueda v:35 ↔ DIN 625 SKF- con escudo Z SKF 625-Z:70
- [Flush]: Rueda v:35 ↔ DIN 625 SKF- con escudo Z SKF 625-Z:71
- [Mate]: DIN 625 SKF- con escudo Z SKF 625-Z:70 ↔ ISO 4014 M5 x 35:28
- [Mate]: DIN 625 SKF- con escudo Z SKF 625-Z:70 ↔ ISO 4014 M5 x 35:28
- [Mate]: ISO 4014 M5 x 35:28 ↔ Buje paraVslot:27
- [Mate]: DIN 625 SKF- con escudo Z SKF 625-Z:71 ↔ Buje paraVslot:27
- [Mate]: ISO 4014 M5 x 35:28 ↔ ISO 4032 M5:29
- [Mate]: ISO 4014 M5 x 35:28 ↔ ISO 7093 A ST 5 - 140 HV - A:39
- [Mate]: Buje paraVslot:27 ↔ ISO 7093 A ST 5 - 140 HV - A:39
- [Mate]: Soporte del primer segmento:2 ↔ ISO 4014 M5 x 35:25
- [Mate]: Soporte del primer segmento:2 ↔ ISO 7093 A ST 5 - 140 HV - A:36
- [Angle] (0 deg): Soporte del primer segmento:2 ↔ ISO 4032 M5:26
- [Mate]: Soporte del primer segmento:2 ↔ ISO 4032 M5:26
- [Mate]: Soporte del primer segmento:2 ↔ ISO 4014 M5 x 35:26
- [Mate]: Soporte del primer segmento:2 ↔ ISO 7093 A ST 5 - 140 HV - A:37
- [Mate]: Soporte del primer segmento:2 ↔ ISO 4032 M5:27
- [Angle] (0 deg): Soporte del primer segmento:2 ↔ ISO 4032 M5:27
- [Mate]: Soporte del primer segmento:2 ↔ ISO 7093 A ST 5 - 140 HV - A:39
- [Mate]: Soporte del primer segmento:2 ↔ ISO 4032 M5:29
- [Angle] (0 deg): Soporte del primer segmento:2 ↔ ISO 4032 M5:29
- [Mate]: Soporte del primer segmento:2 ↔ ISO 7093 A ST 5 - 140 HV - A:38
- [Mate]: Soporte del primer segmento:2 ↔ ISO 4032 M5:28
- [Angle] (0 deg): Soporte del primer segmento:2 ↔ ISO 4032 M5:28
- [Mate]: ISO 4017 M5 x 25:6 ↔ ISO 4032 M5:33
- [Mate]: ISO 4017 M5 x 25:7 ↔ ISO 4032 M5:32
- [Mate]: ISO 4017 M5 x 25:5 ↔ ISO 4032 M5:31
- [Mate]: ISO 4017 M5 x 25:8 ↔ ISO 4032 M5:30
- [Mate]: ISO 4017 M5 x 25:8 ↔ ISO 7089 5:6
- [Mate]: ISO 4017 M5 x 25:5 ↔ ISO 7089 5:5
- [Mate]: ISO 4017 M5 x 25:7 ↔ ISO 7089 5:7
- [Mate]: ISO 4017 M5 x 25:6 ↔ ISO 7089 5:8
- [Mate]: ISO 4032 M5:33 ↔ ISO 7089 5:8
- [Mate]: ISO 4032 M5:32 ↔ ISO 7089 5:7
- [Mate]: ISO 4032 M5:30 ↔ ISO 7089 5:6
- [Mate]: ISO 4032 M5:31 ↔ ISO 7089 5:5
- [Mate]: Soporte del primer segmento:2 ↔ ISO 7089 5:5
- [Mate]: Soporte del primer segmento:2 ↔ ISO 7089 5:6
- [Mate]: Soporte del primer segmento:2 ↔ ISO 7089 5:7
- [Mate]: Soporte del primer segmento:2 ↔ ISO 4017 M5 x 25:5
- [Mate]: Soporte del primer segmento:2 ↔ ISO 4014 M5 x 35:28
- [Mate]: Soporte del primer segmento:2 ↔ ISO 4014 M5 x 35:27
- [Mate]: Soporte del primer segmento:2 ↔ ISO 7089 5:8
- Coincidencia:881 [Mate]: Soporte del primer segmento:2 ↔ Segmento inferior:1
- Coincidencia:882 [Mate]: Soporte del primer segmento:2 ↔ Segmento inferior:1
- Coincidencia:883 [Mate]: Soporte del primer segmento:2 ↔ ISO 4017 M5 x 25:8
- Coincidencia:884 [Mate]: Soporte del primer segmento:2 ↔ ISO 4017 M5 x 25:5
- Coincidencia:885 [Mate]: Soporte del primer segmento:2 ↔ ISO 4017 M5 x 25:7
- Coincidencia:886 [Mate]: Soporte del primer segmento:2 ↔ ISO 4017 M5 x 25:6
- Coincidencia:887 [Mate]: ISO 4017 M5 x 25:5 ↔ Segmento inferior:1
- Ángulo:24 [Angle] (0 deg): ISO 4017 M5 x 25:5 ↔ Segmento inferior:1
- Ángulo:25 [Angle] (0 deg): ISO 4017 M5 x 25:8 ↔ Segmento inferior:1
- Coincidencia:888 [Mate]: Soporte del primer segmento:2 ↔ Segmento inferior:1
- Ángulo:26 [Angle] (0 deg): ISO 4017 M5 x 25:6 ↔ Segmento inferior:1
- Ángulo:27 [Angle] (0 deg): ISO 4017 M5 x 25:7 ↔ Segmento inferior:1
- Coincidencia:889 [Mate]: ISO 4017 M5 x 25:7 ↔ Segmento inferior:1
- Coincidencia:890 [Mate]: ISO 4017 M5 x 25:6 ↔ Segmento inferior:1
- Coincidencia:891 [Mate]: ISO 4017 M5 x 25:8 ↔ Segmento inferior:1
- Ángulo:28 [Angle] (0 deg): Poste:1 ↔ Segmento inferior:1
- Ángulo:29 [Angle] (0 deg): Poste:1 ↔ Soporte del primer segmento:2
- Coincidencia:892 [Mate]: Segmento inferior:1 ↔ Nema+17+Motor+Assembled:5
- Coincidencia:893 [Mate]: Segmento inferior:1 ↔ Nema+17+Motor+Assembled:5
- Coincidencia:894 [Mate]: Segmento inferior:1 ↔ Nema+17+Motor+Assembled:5
- Coincidencia:895 [Mate]: DIN 625 SKF- con escudo Z SKF 608-Z:5 ↔ Segmento inferior:1
- Nivelación:107 [Flush]: DIN 625 SKF- con escudo Z SKF 608-Z:5 ↔ Segmento inferior:1
- Coincidencia:896 [Mate]: Segmento inferior:1 ↔ Primer segmento - superior v1.2:1
- Coincidencia:897 [Mate]: DIN 625 SKF- con escudo Z SKF 608-Z:5 ↔ Primer segmento - superior v1.2:1
- Coincidencia:898 [Mate]: Segmento inferior:1 ↔ Primer segmento - superior v1.2:1
- Coincidencia:899 [Mate]: DIN 625 SKF- con escudo Z SKF 608-Z:6 ↔ Primer segmento - superior v1.2:1
- Nivelación:108 [Flush]: DIN 625 SKF- con escudo Z SKF 608-Z:6 ↔ Primer segmento - superior v1.2:1
- Coincidencia:900 [Mate]: DIN 625 SKF- con escudo Z SKF 608-Z:9 ↔ Segmento inferior:1
- Nivelación:109 [Flush]: DIN 625 SKF- con escudo Z SKF 608-Z:9 ↔ Segmento inferior:1
- Coincidencia:901 [Mate]: ISO 2338 8 h8 x 40:3 ↔ DIN 625 SKF- con escudo Z SKF 608-Z:6
- Nivelación:110 [Flush]: ISO 2338 8 h8 x 40:3 ↔ DIN 625 SKF- con escudo Z SKF 608-Z:6
- Coincidencia:903 [Mate]: Engranaje para nema 17:4 ↔ Nema+17+Motor+Assembled:5
- Coincidencia:904 [Mate]: Primer segmento - superior v1.2:1 ↔ ISO 7045 H M3 x 8 - 4.8 - H:14
- Coincidencia:905 [Mate]: Primer segmento - superior v1.2:1 ↔ ISO 7045 H M3 x 8 - 4.8 - H:16
- Coincidencia:906 [Mate]: Primer segmento - superior v1.2:1 ↔ ISO 7045 H M3 x 8 - 4.8 - H:18
- Coincidencia:907 [Mate]: Primer segmento - superior v1.2:1 ↔ ISO 7045 H M3 x 8 - 4.8 - H:19
- Coincidencia:908 [Mate]: Primer segmento - superior v1.2:1 ↔ ISO 7045 H M3 x 8 - 4.8 - H:17
- Coincidencia:909 [Mate]: Primer segmento - superior v1.2:1 ↔ ISO 7045 H M3 x 8 - 4.8 - H:15
- Coincidencia:910 [Mate]: Primer segmento - superior v1.2:1 ↔ ISO 7045 H M3 x 8 - 4.8 - H:14
- Coincidencia:911 [Mate]: Primer segmento - superior v1.2:1 ↔ ISO 7045 H M3 x 8 - 4.8 - H:15
- Coincidencia:912 [Mate]: Primer segmento - superior v1.2:1 ↔ ISO 7045 H M3 x 8 - 4.8 - H:16
- Coincidencia:913 [Mate]: Primer segmento - superior v1.2:1 ↔ ISO 7045 H M3 x 8 - 4.8 - H:18
- Coincidencia:914 [Mate]: Primer segmento - superior v1.2:1 ↔ ISO 7045 H M3 x 8 - 4.8 - H:19
- Coincidencia:915 [Mate]: Primer segmento - superior v1.2:1 ↔ ISO 7045 H M3 x 8 - 4.8 - H:17
- Coincidencia:916 [Mate]: Primer segmento - superior v1.2:1 ↔ JIS B 1521 6805 25x37x7:3
- Nivelación:112 [Flush]: Primer segmento - superior v1.2:1 ↔ JIS B 1521 6805 25x37x7:3
- Coincidencia:917 [Mate]: ISO 2338 8 h8 x 40:3 ↔ Engrajane doble - primer segmento:2
- Coincidencia:919 [Mate]: JIS B 1521 6805 25x37x7:3 ↔ Engranaje simple - primer segmento:1
- Nivelación:113 [Flush]: Engrajane doble - primer segmento:2 ↔ Engranaje simple - primer segmento:1
- Nivelación:114 [Flush]: Engrajane doble - primer segmento:2 ↔ Engranaje para nema 17:4
- Coincidencia:929 [Mate]: Engranaje simple - primer segmento:1 ↔ ISO 4017 M4 x 40:4
- Coincidencia:930 [Mate]: Engranaje simple - primer segmento:1 ↔ ISO 4017 M4 x 40:2
- Coincidencia:931 [Mate]: Engranaje simple - primer segmento:1 ↔ ISO 4017 M4 x 40:1
- Coincidencia:932 [Mate]: Engranaje simple - primer segmento:1 ↔ ISO 4017 M4 x 40:3
- Coincidencia:933 [Mate]: ISO 4017 M4 x 40:4 ↔ ISO 4032 M4:3
- Coincidencia:934 [Mate]: ISO 4017 M4 x 40:2 ↔ ISO 4032 M4:4
- Coincidencia:935 [Mate]: ISO 4017 M4 x 40:1 ↔ ISO 4032 M4:1